# Autodesk Inventor assembly: PrzekladniaLewa
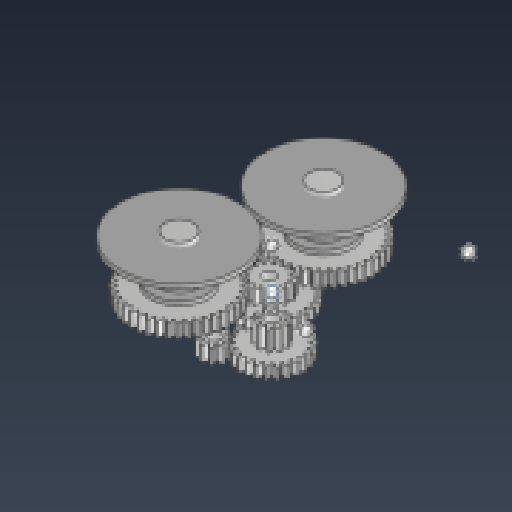
[picture p0: Inventor's stored thumbnail of the model, 512x512]
Saved by Autodesk Inventor 2023 (Build 270158000, 158)
## iProperties
Created: 2022-03-16
Part Number: PrzekladniaLewa
Material: Ogólny
Document SubType Name: Assembly
Designer: Michał
Mass: 30.2365 g
Surface Area: 69.5934 cm^2
Volume: 4.93321 cm^3
Density: 6.12918 g/cm^3
Author: Michał
## Documents named in this file (11)
- D:\tech\robotyka\robots\evangelion\inventor-project\LeftGearbox.iam
- D:\tech\robotyka\robots\evangelion\inventor-project\LeftGearbox\Design Accelerator\Przekładnia walcowa14.ipt
- D:\tech\robotyka\robots\evangelion\inventor-project\LeftGearbox\Design Accelerator\Przekładnia walcowa22.ipt
- D:\tech\robotyka\robots\evangelion\inventor-project\LeftGearbox\Design Accelerator\Przekładnia walcowa23.ipt
- D:\tech\robotyka\robots\evangelion\inventor-project\LeftGearbox\Design Accelerator\Przekładnia walcowa24.ipt
- D:\tech\robotyka\robots\evangelion\inventor-project\LeftGearbox\Design Accelerator\Przekładnia walcowa12.ipt
- D:\tech\robotyka\robots\evangelion\inventor-project\LeftGearbox\Design Accelerator\Przekładnia walcowa13.ipt
- D:\tech\robotyka\robots\evangelion\inventor-project\oponka-dziurawa-prototyp\wheel.ipt
- D:\tech\robotyka\robots\evangelion\inventor-project\oponka-dziurawa-prototyp\ball-bearing-6x10x3.ipt
- D:\tech\robotyka\robots\evangelion\inventor-project\Lozysko GFM-0608-04.ipt
- D:\tech\robotyka\robots\evangelion\inventor-project\Lozysko GFM-0608-2.ipt
## Components (15 placed, 6 different names)
1. Przekładnia walcowa1:3 — Tangent:1, Rotation:1, Flush:1, Mate:11, Mate:12, Flush:2, Mate:13, Mate:14, Mate:15, Mate:16
2. Przekładnia walcowa1:1 — Mate:8, Mate:9, Rotation:4, Tangent:3, Rotation:5, Tangent:4, Rotation:6
3. Przekładnia walcowa2:1 — Mate:5, Mate:6, Rotation:2, Tangent:2, Rotation:3
4. Przekładnia walcowa2:2 — Mate:7, Tangent:2, Rotation:3, Mate:8, Mate:9, Rotation:4, Mate:10, Mate:21
5. Przekładnia walcowa2:3 — Mate:10, Tangent:3, Rotation:5, Mate:23, Flush:25, Mate:25, Mate:27, Mate:32, Mate:35, Mate:37, Mate:38
6. Przekładnia walcowa1:2 — Tangent:1, Rotation:1, Flush:1, Mate:5, Mate:6, Rotation:2, Mate:7
7. Przekładnia walcowa2:4 — Mate:21, Tangent:4, Rotation:6, Mate:22, Flush:24, Mate:24, Mate:26, Mate:33, Mate:34, Mate:39, Mate:40
8. wheel:1 — Mate:22, Flush:24
9. wheel:2 — Mate:23, Flush:25
10. ball-bearing-6x10x3:1 — Mate:25, Mate:27
11. ball-bearing-6x10x3:2 — Mate:24, Mate:26
12. Lozysko GFM-0608-04:3 — Mate:33, Mate:34
13. Lozysko GFM-0608-04:4 — Mate:32, Mate:35
14. Lozysko GFM-0608-2:1 — Mate:39, Mate:40
15. Lozysko GFM-0608-2:2 — Mate:37, Mate:38
## Relationships (41: Mate 27, RelateRotation 6, Tangent 4, Flush 4)
- Tangent:1: Przekładnia walcowa1:3 ↔ Przekładnia walcowa1:2
- Rotation:1 [RelateRotation] (0.4 ul): Przekładnia walcowa1:3 ↔ Przekładnia walcowa1:2
- Flush:1: Przekładnia walcowa1:3 ↔ Przekładnia walcowa1:2
- Mate:5: Przekładnia walcowa2:1 ↔ Przekładnia walcowa1:2
- Mate:6: Przekładnia walcowa2:1 ↔ Przekładnia walcowa1:2
- Rotation:2 [RelateRotation] (1 ul): Przekładnia walcowa2:1 ↔ Przekładnia walcowa1:2
- Mate:7 (0.1 mm): Przekładnia walcowa2:2 ↔ Przekładnia walcowa1:2
- Tangent:2: Przekładnia walcowa2:1 ↔ Przekładnia walcowa2:2
- Rotation:3 [RelateRotation] (0.333 ul): Przekładnia walcowa2:1 ↔ Przekładnia walcowa2:2
- Mate:8: Przekładnia walcowa1:1 ↔ Przekładnia walcowa2:2
- Mate:9: Przekładnia walcowa1:1 ↔ Przekładnia walcowa2:2
- Rotation:4 [RelateRotation] (0.5 ul): Przekładnia walcowa1:1 ↔ Przekładnia walcowa2:2
- Mate:10 (0.1 mm): Przekładnia walcowa2:2 ↔ Przekładnia walcowa2:3
- Tangent:3: Przekładnia walcowa1:1 ↔ Przekładnia walcowa2:3
- Rotation:5 [RelateRotation] (0.375 ul): Przekładnia walcowa1:1 ↔ Przekładnia walcowa2:3
- Mate:11: Przekładnia walcowa1:3
- Mate:12: Przekładnia walcowa1:3
- Flush:2: Przekładnia walcowa1:3
- Mate:13: Przekładnia walcowa1:3
- Mate:14: Przekładnia walcowa1:3
- Mate:15: Przekładnia walcowa1:3
- Mate:16: Przekładnia walcowa1:3
- Mate:21 (0.1 mm): Przekładnia walcowa2:2 ↔ Przekładnia walcowa2:4
- Tangent:4: Przekładnia walcowa1:1 ↔ Przekładnia walcowa2:4
- Rotation:6 [RelateRotation] (2.667 ul): Przekładnia walcowa1:1 ↔ Przekładnia walcowa2:4
- Mate:22: Przekładnia walcowa2:4 ↔ wheel:1
- Flush:24 (1 mm): Przekładnia walcowa2:4 ↔ wheel:1
- Mate:23: Przekładnia walcowa2:3 ↔ wheel:2
- Flush:25 (1 mm): Przekładnia walcowa2:3 ↔ wheel:2
- Mate:24: Przekładnia walcowa2:4 ↔ ball-bearing-6x10x3:2
- Mate:25: Przekładnia walcowa2:3 ↔ ball-bearing-6x10x3:1
- Mate:26 (0.1 mm): Przekładnia walcowa2:4 ↔ ball-bearing-6x10x3:2
- Mate:27 (0.1 mm): Przekładnia walcowa2:3 ↔ ball-bearing-6x10x3:1
- Mate:32: Przekładnia walcowa2:3 ↔ Lozysko GFM-0608-04:4
- Mate:33: Przekładnia walcowa2:4 ↔ Lozysko GFM-0608-04:3
- Mate:34: Przekładnia walcowa2:4 ↔ Lozysko GFM-0608-04:3
- Mate:35: Przekładnia walcowa2:3 ↔ Lozysko GFM-0608-04:4
- Mate:37: Przekładnia walcowa2:3 ↔ Lozysko GFM-0608-2:2
- Mate:38: Przekładnia walcowa2:3 ↔ Lozysko GFM-0608-2:2
- Mate:39: Przekładnia walcowa2:4 ↔ Lozysko GFM-0608-2:1
- Mate:40: Przekładnia walcowa2:4 ↔ Lozysko GFM-0608-2:1
